# Autodesk Inventor assembly: ASY Disk Micro filter v2.0
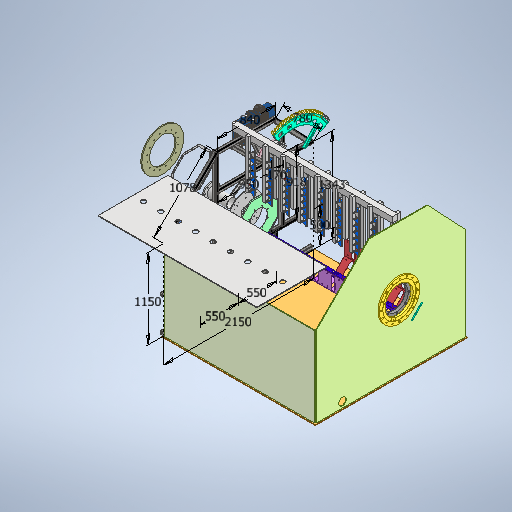
[picture p0: Inventor's stored thumbnail of the model, 512x512]
Saved by Autodesk Inventor 2026 (Build 300175000, 175)
## iProperties
Created: 2023-08-31
Part Number: ASY Disk Micro filter v2.0
Document SubType Name: Assembly
Designer: admin
Stock Number: Дисковый_Фильтр
Author: admin
## Documents named in this file (38)
- C:\Users\pokla\Documents\Inventor\ДФО\ДМФ\DMF-Disk-Micro-Filter\ASY 000 ДМФ Disk Micro filter v2.0.iam
- C:\Users\pokla\Documents\Inventor\ДФО\ДМФ\DMF-Disk-Micro-Filter\Left wall v2.0.ipt
- C:\Users\pokla\Documents\Inventor\ДФО\ДМФ\DMF-Disk-Micro-Filter\Wall right v2.0.ipt
- C:\Users\pokla\Documents\Inventor\ДФО\ДМФ\DMF-Disk-Micro-Filter\DF1.03 Wall bottom v2.0.ipt
- C:\Users\pokla\Documents\Inventor\ДФО\ДМФ\DMF-Disk-Micro-Filter\DF1.04 Wall face v2.0.ipt
- C:\Users\pokla\Documents\Inventor\ДФО\ДМФ\DMF-Disk-Micro-Filter\ДМФ 021 кольцо прижимное нос v2.0.ipt
- C:\Users\pokla\Documents\Inventor\ДФО\ДМФ\DMF-Disk-Micro-Filter\ДМФ 000 размеры v2.0.ipt
- C:\Users\pokla\Documents\Inventor\ДФО\ДМФ\DMF-Disk-Micro-Filter\ДМФ 032 крышка Нос v2.0.ipt
- C:\Users\pokla\Documents\Inventor\ДФО\ДМФ\DMF-Disk-Micro-Filter\ДМФ 091 Постель НОС v2.0.ipt
- C:\Users\pokla\Documents\Inventor\ДФО\ДМФ\DMF-Disk-Micro-Filter\ДМФ 022 кольцо прижимное корма v2.0.ipt
- C:\Users\pokla\Documents\Inventor\ДФО\ДМФ\DMF-Disk-Micro-Filter\ДМФ 093 Постель КОРМА v2.0.ipt
- C:\Users\pokla\Documents\Inventor\ДФО\ДМФ\DMF-Disk-Micro-Filter\ДМФ 092 Коромысло КОРМА v2.0.ipt
- C:\Users\pokla\Documents\Inventor\ДФО\ДМФ\DMF-Disk-Micro-Filter\ДМФ 055 труба илоотвода v2.0.ipt
- C:\Users\pokla\Documents\Inventor\ДФО\ДМФ\DMF-Disk-Micro-Filter\ДМФ 033 держатель лотка v2.0.ipt
- C:\Users\pokla\Documents\Inventor\ДФО\ДМФ\DMF-Disk-Micro-Filter\ASY ДМФ лоток 050 илоотвод v2.0.iam
- C:\Users\pokla\Documents\Inventor\ДФО\ДМФ\DMF-Disk-Micro-Filter\ДМФ 092 Коромысло НОС v2.0.ipt
- C:\Users\pokla\Documents\Inventor\ДФО\ДМФ\DMF-Disk-Micro-Filter\ДМФ 066 Гребенка v2.0.ipt
- C:\Users\pokla\Documents\Inventor\ДФО\ДМФ\DMF-Disk-Micro-Filter\ДМФ 025 кольцо прижимное корма наружное v2.0.ipt
- C:\Users\pokla\Documents\Inventor\ДФО\ДМФ\DMF-Disk-Micro-Filter\ДМФ 067 крышка v2.0.ipt
- C:\Users\pokla\Documents\Inventor\ДФО\ДМФ\DMF-Disk-Micro-Filter\ДМФ 081 труба форсунки v2.0.ipt
- C:\Users\pokla\Documents\Inventor\ДФО\ДМФ\DMF-Disk-Micro-Filter\ASY Обрешетка лицевая стенка.iam
- C:\Users\pokla\Documents\Inventor\ДФО\ДМФ\DMF-Disk-Micro-Filter\ASY Консоль под двигатель вед. шестерни.iam
- C:\Users\pokla\Documents\Inventor\ДФО\ДМФ\DMF-Disk-Micro-Filter\Вал ведущей шестерни.ipt
- C:\Users\pokla\Documents\Inventor\ДФО\ДМФ\DMF-Disk-Micro-Filter\Корпусный подшипник D35.ipt
- C:\Users\pokla\Documents\Inventor\ДФО\ДМФ\DMF-Disk-Micro-Filter\Мотор-редуктор NMRV 090(80B5).ipt
- C:\Users\pokla\Documents\Inventor\ДФО\ДМФ\DMF-Disk-Micro-Filter\DMF pancake.ipt
- C:\Users\pokla\Documents\Inventor\ДФО\ДМФ\DMF-Disk-Micro-Filter\Нога для постели.ipt
- C:\Users\pokla\Documents\Inventor\ДФО\ДМФ\DMF-Disk-Micro-Filter\Нога для постели №2.ipt
- C:\Users\pokla\Documents\Inventor\ДФО\ДМФ\DMF-Disk-Micro-Filter\ДМФ 092 Постель НОС v2.0.ipt
- C:\Users\pokla\Documents\Inventor\ДФО\ДМФ\DMF-Disk-Micro-Filter\ДМФ 094 Постель НОС крепление v2.0.ipt
- C:\Users\pokla\Documents\Inventor\ДФО\ДМФ\DMF-Disk-Micro-Filter\DMF Hat 2.0.ipt
- C:\Users\pokla\Documents\Inventor\ДФО\ДМФ\DMF-Disk-Micro-Filter\DMF Flange exit 2.0.ipt
- C:\Users\pokla\Documents\Inventor\ДФО\ДМФ\DMF-Disk-Micro-Filter\Барабан v2.1\ASY ДМФ 0100 Барабан v2.1.iam
- C:\Users\pokla\Documents\Inventor\ДФО\ДМФ\DMF-Disk-Micro-Filter\Барабан v2.1\DMF flange small gear.ipt
- C:\Users\pokla\Documents\Inventor\ДФО\ДМФ\DMF-Disk-Micro-Filter\Барабан v2.1\DMF small gear.ipt
- C:\Users\pokla\Documents\Inventor\ДФО\ДМФ\DMF-Disk-Micro-Filter\DMF Support ring tail.ipt
- C:\Users\pokla\Documents\Inventor\ДФО\ДМФ\DMF-Disk-Micro-Filter\Промывка Алексенко\Промывка.iam
- C:\Users\pokla\Documents\Inventor\ДФО\ДМФ\DMF-Disk-Micro-Filter\DMF 082 коллектор болванка.ipt
## Components (52 placed, 38 different names)
1. ДМФ 000 размеры v2.0.ipt:1
2. Left wall v2.0.ipt:1 — Заподлицо:4, Совмещение:1, Заподлицо:6, Заподлицо:7, Заподлицо:9, Совмещение:4, Заподлицо:26, Заподлицо:27, Совмещение:25, Жесткий:16, Жесткий:27
3. Wall right v2.0.ipt:1 — Заподлицо:23, Заподлицо:24, Жесткий:16, Жесткий:32, Совмещение:32, Совмещение:33
4. DF1.03 Wall bottom v2.0.ipt:1 — Совмещение:1, Заподлицо:6, Заподлицо:7, Совмещение:3, Заподлицо:11, Совмещение:24, Совмещение:30
5. DF1.04 Wall face v2.0.ipt:1 — Заподлицо:9, Совмещение:3, Совмещение:4, Заподлицо:10, Угол:1
6. ДМФ 021 кольцо прижимное нос v2.0.ipt:1
7. ДМФ 032 крышка Нос v2.0.ipt:1
8. ДМФ 091 Постель НОС v2.0.ipt:1
9. ДМФ 022 кольцо прижимное корма v2.0.ipt:1
10. ДМФ 093 Постель КОРМА v2.0.ipt:1
11. ДМФ 092 Коромысло КОРМА v2.0.ipt:1
12. ДМФ 055 труба илоотвода v2.0.ipt:1 — Жесткий:26, Цилиндрический:30
13. ДМФ 033 держатель лотка v2.0.ipt:1
14. ASY ДМФ лоток 050 илоотвод v2.0.iam:1 [sub-assembly]
15. ДМФ 092 Коромысло НОС v2.0.ipt:1
16. ДМФ 066 Гребенка v2.0.ipt:1 — Заподлицо:22, Угол:1, Совмещение:24
17. ДМФ 025 кольцо прижимное корма наружное v2.0.ipt:1
18. ДМФ 067 крышка v2.0.ipt:1 — Заподлицо:23, Заподлицо:24
19. ASY Обрешетка лицевая стенка.iam:1 [sub-assembly] — Заподлицо:26, Заподлицо:27, Совмещение:25, Совмещение:26, Заподлицо:28, Заподлицо:30, Заподлицо:34
20. ASY Консоль под двигатель вед. шестерни.iam:1 [sub-assembly] — Совмещение:26, Заподлицо:28, Заподлицо:30, Совмещение:28, Заподлицо:31, Заподлицо:32, Заподлицо:33, Совмещение:31
21. Вал ведущей шестерни.ipt:1 — Жесткий:30, Жесткий:31
22. Корпусный подшипник D35.ipt:1 — Заподлицо:33, Совмещение:31, Заподлицо:34
23. Мотор-редуктор NMRV 090(80B5).ipt:1 — Совмещение:28, Заподлицо:31, Жесткий:30, Заподлицо:32
24. DMF pancake.ipt:1 — Жесткий:27, Жесткий:28
25. Нога для постели.ipt:1
26. Нога для постели №2.ipt:1
27. ДМФ 092 Постель НОС v2.0.ipt:1
28. ДМФ 094 Постель НОС крепление v2.0.ipt:2
29. DMF Hat 2.0.ipt:1 — Жесткий:28, Цилиндрический:30
30. DMF Flange exit 2.0.ipt:1 — Жесткий:26
31. ASY ДМФ 0100 Барабан v2.1:1 [sub-assembly] — С поворотом:17, С поворотом:18
32. flange small gear:1
33. DMF small gear:1 — Жесткий:31
34. DMF Support ring tail:1 — Жесткий:32, С поворотом:17, С поворотом:18
35. Промывка:1 [sub-assembly]
36. DMF 082 коллектор болванка:1 — Совмещение:32, Совмещение:33, Жесткий:33, Жесткий:34
37. ДМФ 081 труба форсунки v2.0:2 — Жесткий:34
38. ДМФ 081 труба форсунки v2.0.ipt:1 — Жесткий:33
39. ДМФ 081 труба форсунки v2.0:3
40. ДМФ 081 труба форсунки v2.0:4
41. ДМФ 081 труба форсунки v2.0:5
42. ДМФ 081 труба форсунки v2.0:6
43. ДМФ 081 труба форсунки v2.0:7
44. ДМФ 081 труба форсунки v2.0:8
45. ДМФ 081 труба форсунки v2.0:9
46. ДМФ 081 труба форсунки v2.0:10
47. ДМФ 081 труба форсунки v2.0:11
48. ДМФ 081 труба форсунки v2.0:12
49. ДМФ 081 труба форсунки v2.0:13
50. ДМФ 081 труба форсунки v2.0:14
51. ДМФ 081 труба форсунки v2.0:15
52. ДМФ 081 труба форсунки v2.0:16
## Component patterns: (8 elements, first: ДМФ 081 труба форсунки v2.0:2 + ДМФ 081 труба форсунки v2.0.ipt:1)
## Relationships (42: Flush 17, Mate 12, WeldJoint 9, RevoluteJoint 2, Angle 1, CylindricalJoint 1)
- Заподлицо:4 [Flush]: Left wall v2.0.ipt:1
- Совмещение:1 [Mate]: Left wall v2.0.ipt:1 ↔ DF1.03 Wall bottom v2.0.ipt:1
- Заподлицо:6 [Flush] (15 mm): Left wall v2.0.ipt:1 ↔ DF1.03 Wall bottom v2.0.ipt:1
- Заподлицо:7 [Flush] (25 mm): Left wall v2.0.ipt:1 ↔ DF1.03 Wall bottom v2.0.ipt:1
- Заподлицо:9 [Flush]: Left wall v2.0.ipt:1 ↔ DF1.04 Wall face v2.0.ipt:1
- Совмещение:3 [Mate]: DF1.03 Wall bottom v2.0.ipt:1 ↔ DF1.04 Wall face v2.0.ipt:1
- Совмещение:4 [Mate]: Left wall v2.0.ipt:1 ↔ DF1.04 Wall face v2.0.ipt:1
- Заподлицо:10 [Flush]: DF1.04 Wall face v2.0.ipt:1
- Заподлицо:11 [Flush]: DF1.03 Wall bottom v2.0.ipt:1
- [Mate]: ASY ДМФ лоток 050 илоотвод v2.0.iam:1
- Заподлицо:22 [Flush]: ДМФ 066 Гребенка v2.0.ipt:1
- Угол:1 [Angle] (180 deg): DF1.04 Wall face v2.0.ipt:1 ↔ ДМФ 066 Гребенка v2.0.ipt:1
- Совмещение:24 [Mate]: DF1.03 Wall bottom v2.0.ipt:1 ↔ ДМФ 066 Гребенка v2.0.ipt:1
- Заподлицо:23 [Flush]: Wall right v2.0.ipt:1 ↔ ДМФ 067 крышка v2.0.ipt:1
- Заподлицо:24 [Flush] (-50 mm): Wall right v2.0.ipt:1 ↔ ДМФ 067 крышка v2.0.ipt:1
- Заподлицо:26 [Flush]: Left wall v2.0.ipt:1 ↔ ASY Обрешетка лицевая стенка.iam:1
- Заподлицо:27 [Flush]: Left wall v2.0.ipt:1 ↔ ASY Обрешетка лицевая стенка.iam:1
- Совмещение:25 [Mate]: Left wall v2.0.ipt:1 ↔ ASY Обрешетка лицевая стенка.iam:1
- Совмещение:26 [Mate]: ASY Обрешетка лицевая стенка.iam:1 ↔ ASY Консоль под двигатель вед. шестерни.iam:1
- Заподлицо:28 [Flush]: ASY Обрешетка лицевая стенка.iam:1 ↔ ASY Консоль под двигатель вед. шестерни.iam:1
- Жесткий:16 [WeldJoint] (2160 mm): Left wall v2.0.ipt:1 ↔ Wall right v2.0.ipt:1
- Заподлицо:30 [Flush]: ASY Обрешетка лицевая стенка.iam:1 ↔ ASY Консоль под двигатель вед. шестерни.iam:1
- Совмещение:28 [Mate]: ASY Консоль под двигатель вед. шестерни.iam:1 ↔ Мотор-редуктор NMRV 090(80B5).ipt:1
- Заподлицо:31 [Flush]: ASY Консоль под двигатель вед. шестерни.iam:1 ↔ Мотор-редуктор NMRV 090(80B5).ipt:1
- Совмещение:30 [Mate]: DF1.03 Wall bottom v2.0.ipt:1
- Жесткий:26 [WeldJoint]: ДМФ 055 труба илоотвода v2.0.ipt:1 ↔ DMF Flange exit 2.0.ipt:1
- Жесткий:27 [WeldJoint]: Left wall v2.0.ipt:1 ↔ DMF pancake.ipt:1
- Жесткий:28 [WeldJoint]: DMF pancake.ipt:1 ↔ DMF Hat 2.0.ipt:1
- Цилиндрический:30 [CylindricalJoint]: ДМФ 055 труба илоотвода v2.0.ipt:1 ↔ DMF Hat 2.0.ipt:1
- Жесткий:30 [WeldJoint] (-30 mm): Вал ведущей шестерни.ipt:1 ↔ Мотор-редуктор NMRV 090(80B5).ipt:1
- Заподлицо:32 [Flush] (47 mm): ASY Консоль под двигатель вед. шестерни.iam:1 ↔ Мотор-редуктор NMRV 090(80B5).ipt:1
- Жесткий:31 [WeldJoint]: Вал ведущей шестерни.ipt:1 ↔ DMF small gear:1
- Заподлицо:33 [Flush] (66.5 mm): ASY Консоль под двигатель вед. шестерни.iam:1 ↔ Корпусный подшипник D35.ipt:1
- Совмещение:31 [Mate] (55.4 mm): ASY Консоль под двигатель вед. шестерни.iam:1 ↔ Корпусный подшипник D35.ipt:1
- Заподлицо:34 [Flush]: ASY Обрешетка лицевая стенка.iam:1 ↔ Корпусный подшипник D35.ipt:1
- Жесткий:32 [WeldJoint]: Wall right v2.0.ipt:1 ↔ DMF Support ring tail:1
- С поворотом:17 [RevoluteJoint]: ASY ДМФ 0100 Барабан v2.1:1 ↔ DMF Support ring tail:1
- С поворотом:18 [RevoluteJoint]: ASY ДМФ 0100 Барабан v2.1:1 ↔ DMF Support ring tail:1
- Совмещение:32 [Mate]: Wall right v2.0.ipt:1 ↔ DMF 082 коллектор болванка:1
- Совмещение:33 [Mate] (20 mm): Wall right v2.0.ipt:1 ↔ DMF 082 коллектор болванка:1
- Жесткий:33 [WeldJoint]: DMF 082 коллектор болванка:1 ↔ ДМФ 081 труба форсунки v2.0.ipt:1
- Жесткий:34 [WeldJoint] (-280 mm): DMF 082 коллектор болванка:1 ↔ ДМФ 081 труба форсунки v2.0:2
